# Autodesk Inventor assembly: 16mm_Tube_Connector
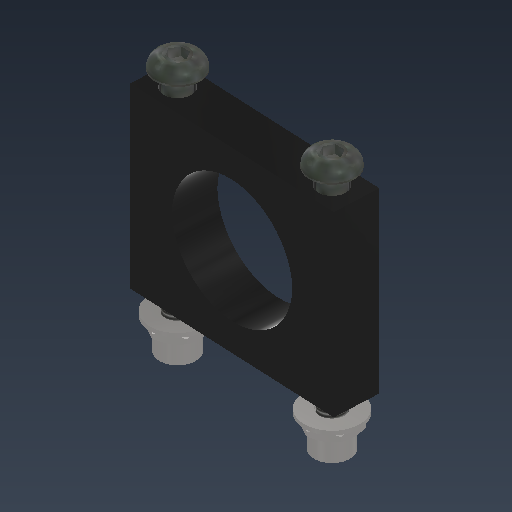
[picture p0: Inventor's stored thumbnail of the model, 512x512]
Saved by Autodesk Inventor 2024.1 (Build 281209000, 209)
## iProperties
Created: 2023-12-05
Part Number: 16mm_Tube_Connector
Document SubType Name: Assembly
Designer: dzw04
Mass: 6.88642 g
Surface Area: 32.9947 cm^2
Volume: 2.47379 cm^3
Density: 2.78375 g/cm^3
Author: dzw04
## Documents named in this file (6)
- C:\Users\dzw04\OneDrive - Saxion\General - Mechatronica Lectoraat LMECH LED\Database ARG\Component_Database\SARAX\01. CAD\01. 3D_Drawing\02. Sub_Assemblies\Landing_Gear\02. Sub_Assemblies\16mm_Tube_Connector.iam
- C:\Users\dzw04\OneDrive - Saxion\General - Mechatronica Lectoraat LMECH LED\Database ARG\Component_Database\SARAX\01. CAD\01. 3D_Drawing\02. Sub_Assemblies\Landing_Gear\01. Parts\16mm_Tube_Connecotor_Holybro.ipt
- C:\Users\dzw04\OneDrive - Saxion\General - Mechatronica Lectoraat LMECH LED\Database ARG\Component_Database\SARAX\01. CAD\01. 3D_Drawing\01. Parts\en-US\ISO 7380-1\ISO 7380-1 - M3 x 30.ipt
- C:\Users\dzw04\OneDrive - Saxion\General - Mechatronica Lectoraat LMECH LED\Database ARG\Component_Database\SARAX\01. CAD\01. 3D_Drawing\01. Parts\en-US\ISO 7089\ISO 7089 - 3 - 140 HV(1).ipt
- C:\Users\dzw04\OneDrive - Saxion\General - Mechatronica Lectoraat LMECH LED\Database ARG\Component_Database\SARAX\01. CAD\01. 3D_Drawing\01. Parts\en-US\ISO 10511\ISO 10511 - M3.ipt
- C:\Users\dzw04\OneDrive - Saxion\General - Mechatronica Lectoraat LMECH LED\Database ARG\Component_Database\SARAX\01. CAD\01. 3D_Drawing\Parameters.xlsx
## Components (8 placed, 4 different names)
1. 16mm_Tube_Connecotor_Holybro:1 — Mate:1, Flush:1, Flush:2, Mate:4, Mate:6, Mate:10, Mate:11
2. 16mm_Tube_Connecotor_Holybro:2 — Mate:1, Flush:1, Flush:2, Mate:2, Mate:3
3. ISO 7380-1 M3 x 30:1 — Mate:3, Mate:11, Mate:12, Mate:13
4. ISO 7089 3:1 — Mate:4, Mate:5, Mate:13
5. DIN EN ISO 10511 M3:1 — Mate:5, Mate:12
6. ISO 7380-1 M3 x 30:2 — Mate:2, Mate:8, Mate:9, Mate:10
7. ISO 7089 3:2 — Mate:6, Mate:7, Mate:9
8. DIN EN ISO 10511 M3:2 — Mate:7, Mate:8
## Relationships (15: Mate 13, Flush 2)
- Mate:1: 16mm_Tube_Connecotor_Holybro:1 ↔ 16mm_Tube_Connecotor_Holybro:2
- Flush:1: 16mm_Tube_Connecotor_Holybro:1 ↔ 16mm_Tube_Connecotor_Holybro:2
- Flush:2: 16mm_Tube_Connecotor_Holybro:1 ↔ 16mm_Tube_Connecotor_Holybro:2
- Mate:2 (2 mm): 16mm_Tube_Connecotor_Holybro:2 ↔ ISO 7380-1 M3 x 30:2
- Mate:3 (2 mm): 16mm_Tube_Connecotor_Holybro:2 ↔ ISO 7380-1 M3 x 30:1
- Mate:4 (2 mm): 16mm_Tube_Connecotor_Holybro:1 ↔ ISO 7089 3:1
- Mate:5: ISO 7089 3:1 ↔ DIN EN ISO 10511 M3:1
- Mate:6 (2 mm): 16mm_Tube_Connecotor_Holybro:1 ↔ ISO 7089 3:2
- Mate:7: ISO 7089 3:2 ↔ DIN EN ISO 10511 M3:2
- Mate:8: ISO 7380-1 M3 x 30:2 ↔ DIN EN ISO 10511 M3:2
- Mate:9: ISO 7380-1 M3 x 30:2 ↔ ISO 7089 3:2
- Mate:10: 16mm_Tube_Connecotor_Holybro:1 ↔ ISO 7380-1 M3 x 30:2
- Mate:11: 16mm_Tube_Connecotor_Holybro:1 ↔ ISO 7380-1 M3 x 30:1
- Mate:12: ISO 7380-1 M3 x 30:1 ↔ DIN EN ISO 10511 M3:1
- Mate:13: ISO 7380-1 M3 x 30:1 ↔ ISO 7089 3:1
## Named parameters: NumberOfArms = 4, RotorToRotor = 900 mm, MountToMotorCenter = 0 mm, ArmPosition = 5 deg, LoadpipeLength = 450 mm, NumberOfBatterys = 2, BatteryLength = 200 mm, BatteryWidth = 62 mm, BatteryHeight = 76 mm, ThicknessBodyOuterPlate = 2 mm, ThicknessBodyCenterPlate = 2 mm, ThicknessLegLoadpipePlate = 2 mm, ThicknessBatteryTray = 2 mm, ThicknessBatteryTopTray = 1 mm, LandingGearHeight = 400 mm, LandingGearStabilityBar = 525 mm, LandingGearRod = 390 mm, StartAngleArm = 45 deg, MotorMountCenter = 71.5 mm
